# Autodesk Inventor assembly: Wheel Assembly
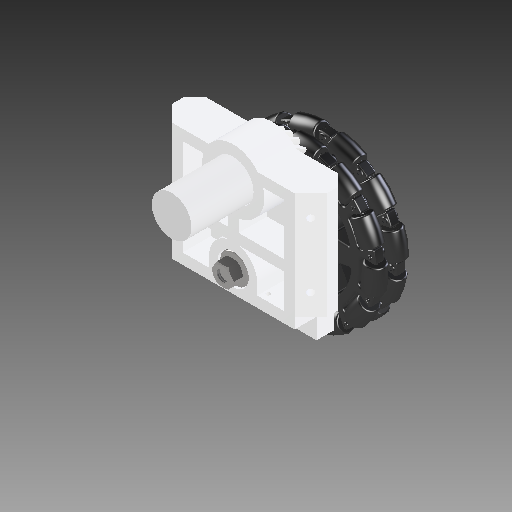
[picture p0: Inventor's stored thumbnail of the model, 512x512]
Saved by Autodesk Inventor 2017 (Build 210142000, 142)
## iProperties
Created: 2017-08-01
Part Number: Wheel Assembly
Document SubType Name: Assembly
Designer: Zach
Author: Zach
## Documents named in this file (11)
- C:\Users\Dell\Documents\GitHub\tr1\src\Base\Wheel Assembly\Wheel Assembly.iam
- C:\Users\Dell\Documents\GitHub\tr1\lib\Omni Wheel 6in\217-2585.ipt
- C:\Users\Dell\Documents\GitHub\tr1\lib\28x12x8mm Bearing.ipt
- C:\Users\Dell\Documents\GitHub\tr1\src\Base\Wheel Assembly\WA004.ipt
- C:\Users\Dell\Documents\GitHub\tr1\src\Base\Wheel Assembly\WA002.ipt
- C:\Users\Dell\Documents\GitHub\tr1\lib\AS 1110 - M12 x 100.ipt
- C:\Users\Dell\Documents\GitHub\tr1\lib\ISO 4032 - M12 - ISO.ipt
- C:\Users\Dell\Documents\GitHub\tr1\lib\6mm Mounting Hub.ipt
- C:\Users\Dell\Documents\GitHub\tr1\lib\12V DC Motor\12V DC Motor.iam
- C:\Users\Dell\Documents\GitHub\tr1\src\Base\Wheel Assembly\Small Gear.iam
- C:\Users\Dell\Documents\GitHub\tr1\src\Base\Wheel Assembly\Wheel Assembly\Design Accelerator\Spur Gears3.iam
## Components (11 placed, 10 different names)
1. 217-2585:1 — Mate:34, Mate:79, Mate:83
2. WA004:1 — Mate:17, Mate:18, Mate:19, Mate:20, Mate:34, Mate:42, Mate:56, Mate:57, Mate:67, Mate:68, Mate:69, Mate:70, Mate:74
3. 28x12x8mm Bearing:3 — Mate:19, Mate:20
4. 28x12x8mm Bearing:4 — Mate:17, Mate:18, Mate:46, Mate:84
5. WA002:1 — Mate:80, Mate:81, Mate:82
6. AS 1110 - Metric M12 x 100:1 — Mate:45, Mate:51, Mate:52, Mate:73, Mate:81, Mate:82, Mate:84
7. ISO 4032 M12:1 — Mate:45, Mate:46
8. 6mm Mounting Hub:1 — Mate:56, Mate:57, Mate:75, Mate:77, Mate:78
9. 12V DC Motor:1 [sub-assembly] — Mate:67, Mate:68, Mate:69, Mate:76
10. Small Gear:1 [sub-assembly] — Mate:73, Mate:74, Rotation:1, Mate:79, Mate:80, Mate:83
11. Spur Gears:2 [sub-assembly] — Mate:75, Mate:76, Mate:77, Mate:78, Rotation:1
## Relationships (29: Mate 28, RelateRotation 1)
- Mate:17: WA004:1 ↔ 28x12x8mm Bearing:4
- Mate:18: WA004:1 ↔ 28x12x8mm Bearing:4
- Mate:19: WA004:1 ↔ 28x12x8mm Bearing:3
- Mate:20: WA004:1 ↔ 28x12x8mm Bearing:3
- Mate:34: 217-2585:1 ↔ WA004:1
- Mate:42: WA004:1
- Mate:45: AS 1110 - Metric M12 x 100:1 ↔ ISO 4032 M12:1
- Mate:46: 28x12x8mm Bearing:4 ↔ ISO 4032 M12:1
- Mate:51: AS 1110 - Metric M12 x 100:1
- Mate:52: AS 1110 - Metric M12 x 100:1
- Mate:56: WA004:1 ↔ 6mm Mounting Hub:1
- Mate:57: WA004:1 ↔ 6mm Mounting Hub:1
- Mate:67: WA004:1 ↔ 12V DC Motor:1
- Mate:68: WA004:1 ↔ 12V DC Motor:1
- Mate:69: WA004:1 ↔ 12V DC Motor:1
- Mate:70: WA004:1
- Mate:73: AS 1110 - Metric M12 x 100:1 ↔ Small Gear:1
- Mate:74: WA004:1 ↔ Small Gear:1
- Mate:75: 6mm Mounting Hub:1 ↔ Spur Gears:2
- Mate:76: 12V DC Motor:1 ↔ Spur Gears:2
- Mate:77: 6mm Mounting Hub:1 ↔ Spur Gears:2
- Mate:78: 6mm Mounting Hub:1 ↔ Spur Gears:2
- Rotation:1 [RelateRotation] (0.5135 ul): Small Gear:1 ↔ Spur Gears:2
- Mate:79: 217-2585:1 ↔ Small Gear:1
- Mate:80: WA002:1 ↔ Small Gear:1
- Mate:81: WA002:1 ↔ AS 1110 - Metric M12 x 100:1
- Mate:82: WA002:1 ↔ AS 1110 - Metric M12 x 100:1
- Mate:83: 217-2585:1 ↔ Small Gear:1
- Mate:84: 28x12x8mm Bearing:4 ↔ AS 1110 - Metric M12 x 100:1
